# Autodesk Inventor assembly: sestavaaaaaaa
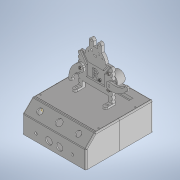
[picture p0: Inventor's stored thumbnail of the model, 180x180]
Saved by Autodesk Inventor 2022 (Build 260153000, 153)
## iProperties
Created: 2022-08-25
Part Number: sestavaaaaaaa
Document SubType Name: Assembly
Designer: Ruslana Zubareva
Author: Ruslana Zubareva
## Documents named in this file (8)
- C:\Users\Ruslana Zubareva\Desktop\sestavaaaaaaa.iam
- C:\Users\Ruslana Zubareva\Desktop\mavac_postava_XD.ipt
- C:\Users\Ruslana Zubareva\Desktop\mavac_krabicka.ipt
- C:\Users\Ruslana Zubareva\Desktop\mavac_vicko.ipt
- C:\Users\Ruslana Zubareva\Desktop\motooor.ipt
- C:\Users\Ruslana Zubareva\Desktop\mavac_ruka_I_know.ipt
- C:\Users\Ruslana Zubareva\Desktop\mavac_ruka_I_know - 2 obycejna.ipt
- C:\Users\Ruslana Zubareva\Documents\Inventor\Content Center Files\R2022\en-US\CNS 4355\CNS 4355 - M 4 x 4.ipt
## Components (9 placed, 7 different names)
1. mavac_krabicka:1 — Mate:1, Mate:2, Mate:3
2. mavac_vicko:1 — Mate:1, Mate:2, Mate:3, Mate:4, Mate:5, Mate:6
3. mavac_postava_XD:1 — Mate:4, Mate:5, Mate:6, Mate:7, Mate:8, Mate:9, Mate:12, Mate:13, Mate:16, Mate:17, Mate:18, Mate:19
4. motooor:1 — Mate:7, Mate:8, Mate:9, Mate:10, Mate:11
5. mavac_ruka_I_know:1 — Mate:10, Mate:11
6. mavac_ruka_I_know - 2 obycejna:1 — Mate:12, Mate:13, Mate:14, Mate:15
7. CNS 4355 M 4 x 4:1 — Mate:14, Mate:15
8. CNS 4355 M 4 x 4:2 — Mate:16, Mate:18
9. CNS 4355 M 4 x 4:3 — Mate:17, Mate:19
## Relationships (19: Mate 19)
- Mate:1: mavac_krabicka:1 ↔ mavac_vicko:1
- Mate:2: mavac_krabicka:1 ↔ mavac_vicko:1
- Mate:3: mavac_krabicka:1 ↔ mavac_vicko:1
- Mate:4: mavac_vicko:1 ↔ mavac_postava_XD:1
- Mate:5: mavac_vicko:1 ↔ mavac_postava_XD:1
- Mate:6: mavac_vicko:1 ↔ mavac_postava_XD:1
- Mate:7: mavac_postava_XD:1 ↔ motooor:1
- Mate:8: mavac_postava_XD:1 ↔ motooor:1
- Mate:9: mavac_postava_XD:1 ↔ motooor:1
- Mate:10: motooor:1 ↔ mavac_ruka_I_know:1
- Mate:11: motooor:1 ↔ mavac_ruka_I_know:1
- Mate:12: mavac_postava_XD:1 ↔ mavac_ruka_I_know - 2 obycejna:1
- Mate:13: mavac_postava_XD:1 ↔ mavac_ruka_I_know - 2 obycejna:1
- Mate:14: mavac_ruka_I_know - 2 obycejna:1 ↔ CNS 4355 M 4 x 4:1
- Mate:15: mavac_ruka_I_know - 2 obycejna:1 ↔ CNS 4355 M 4 x 4:1
- Mate:16: mavac_postava_XD:1 ↔ CNS 4355 M 4 x 4:2
- Mate:17: mavac_postava_XD:1 ↔ CNS 4355 M 4 x 4:3
- Mate:18: mavac_postava_XD:1 ↔ CNS 4355 M 4 x 4:2
- Mate:19: mavac_postava_XD:1 ↔ CNS 4355 M 4 x 4:3
